# Autodesk Inventor assembly: turn
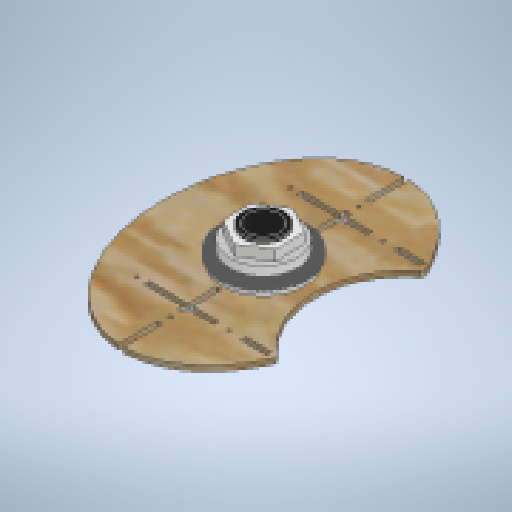
[picture p0: Inventor's stored thumbnail of the model, 512x512]
Saved by Autodesk Inventor 2023.1 (Build 271208000, 208)
## iProperties
Created: 2025-08-10
Part Number: turn
Document SubType Name: Assembly
Designer: DELL
Author: DELL
## Documents named in this file (7)
- C:\Users\DELL\reposGitHub\Cheburashka\Cheburashka_construction\korpus\turn.iam
- C:\Users\DELL\reposGitHub\Cheburashka\Cheburashka_construction\korpus\верхний эллипс туловища.ipt
- C:\Users\DELL\reposGitHub\Cheburashka\Cheburashka_construction\korpus\подш_гл.ipt
- C:\Users\DELL\reposGitHub\Cheburashka\Cheburashka_construction\korpus\сгон.ipt
- C:\Users\DELL\reposGitHub\Cheburashka\Cheburashka_construction\korpus\Деталь2.ipt
- C:\Users\DELL\Downloads\Telegram Desktop\шест1.ipt
- C:\Users\DELL\reposGitHub\Cheburashka\Cheburashka_construction\korpus\Prostavka.ipt
## Components (8 placed, 7 different names)
1. верхний эллипс туловища:1 — Совмещение:1, Совмещение:2, Совмещение:3, Совмещение:13
2. подш_гл:1 — Совмещение:2, Совмещение:3, Совмещение:4
3. сгон:1 — Совмещение:1, Совмещение:5, Совмещение:6, Заподлицо:1, Совмещение:10, Совмещение:14
4. подш_гл:2 — Совмещение:6, Совмещение:11, Совмещение:12, Совмещение:15
5. гайка — Совмещение:4, Совмещение:5, Заподлицо:1
6. Деталь2:2 — Совмещение:10, Совмещение:11
7. шест1:1 — Совмещение:12, Совмещение:16
8. Prostavka:1 — Совмещение:13, Совмещение:14, Совмещение:15, Совмещение:16
## Relationships (14: Mate 13, Flush 1)
- Совмещение:1 [Mate]: верхний эллипс туловища:1 ↔ сгон:1
- Совмещение:2 [Mate]: верхний эллипс туловища:1 ↔ подш_гл:1
- Совмещение:3 [Mate]: верхний эллипс туловища:1 ↔ подш_гл:1
- Совмещение:4 [Mate]: подш_гл:1 ↔ гайка
- Совмещение:5 [Mate]: сгон:1 ↔ гайка
- Совмещение:6 [Mate]: сгон:1 ↔ подш_гл:2
- Заподлицо:1 [Flush]: сгон:1 ↔ гайка
- Совмещение:10 [Mate]: сгон:1 ↔ Деталь2:2
- Совмещение:11 [Mate]: подш_гл:2 ↔ Деталь2:2
- Совмещение:12 [Mate]: подш_гл:2 ↔ шест1:1
- Совмещение:13 [Mate]: верхний эллипс туловища:1 ↔ Prostavka:1
- Совмещение:14 [Mate]: сгон:1 ↔ Prostavka:1
- Совмещение:15 [Mate]: подш_гл:2 ↔ Prostavka:1
- Совмещение:16 [Mate]: шест1:1 ↔ Prostavka:1
